# Autodesk Inventor assembly: Selection_Shaft Weldment
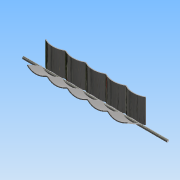
[picture p0: Inventor's stored thumbnail of the model, 180x180]
Saved by Autodesk Inventor 2018.1 (Build 221171000, 171)
## iProperties
Created: 2019-02-11
Part Number: Selection_Shaft Weldment
Document SubType Name: Weldment
Designer: James
Weld Material: Aluminum 6061, Welded
Author: James
## Documents named in this file (4)
- C:\Users\admin\Desktop\Ball Sorting Machine\Ball-Sorting-Machine\Selection Sort\Selection_Shaft Weldment.iam
- C:\Users\admin\Desktop\Ball Sorting Machine\Ball-Sorting-Machine\Selection Sort\Selection_Selector Shaft.ipt
- C:\Users\admin\Desktop\Ball Sorting Machine\Ball-Sorting-Machine\Selection Sort\Selection_Selector Sheet.ipt
- C:\Users\admin\Desktop\Ball Sorting Machine\Ball-Sorting-Machine\Selection Sort\Selection_Selector Sheet Lower.ipt
## Components (3 placed, 3 different names)
1. Selection_Selector Shaft:1 — Flush:1, Flush:2, Flush:3, Tangent:1, Tangent:2, Tangent:3, Tangent:4, Flush:5
2. Selection_Selector Sheet:1 — Flush:4, Tangent:1, Tangent:2, Angle:1, Angle:2
3. Selection_Selector Sheet Lower:1 — Tangent:3, Tangent:4, Flush:5, Angle:2
## Relationships (11: Flush 5, Tangent 4, Angle 2)
- Flush:1: Selection_Selector Shaft:1
- Flush:2: Selection_Selector Shaft:1
- Flush:3: Selection_Selector Shaft:1
- Flush:4: Selection_Selector Sheet:1
- Tangent:1: Selection_Selector Shaft:1 ↔ Selection_Selector Sheet:1
- Tangent:2: Selection_Selector Shaft:1 ↔ Selection_Selector Sheet:1
- Angle:1 (0 deg): Selection_Selector Sheet:1
- Tangent:3: Selection_Selector Shaft:1 ↔ Selection_Selector Sheet Lower:1
- Tangent:4 (1 mm): Selection_Selector Shaft:1 ↔ Selection_Selector Sheet Lower:1
- Flush:5: Selection_Selector Shaft:1 ↔ Selection_Selector Sheet Lower:1
- Angle:2 (-60 deg): Selection_Selector Sheet:1 ↔ Selection_Selector Sheet Lower:1
